# Autodesk Inventor assembly: Total
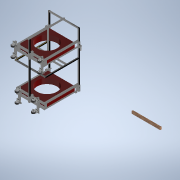
[picture p0: Inventor's stored thumbnail of the model, 180x180]
Saved by Autodesk Inventor 2022 (Build 260153000, 153)
## iProperties
Created: 2022-03-28
Part Number: Total
Document SubType Name: Assembly
Designer: aarco
Author: aarco
## Documents named in this file (14)
- C:\Users\dovalle\OneDrive - ALTER TECHNOLOGY TÜV NORD, S.A.U\Escritorio\IDOM\REV_3\Total.iam
- C:\Users\dovalle\OneDrive - ALTER TECHNOLOGY TÜV NORD, S.A.U\Escritorio\IDOM\REV_3\SoporteBobina_1.iam
- C:\Users\dovalle\OneDrive - ALTER TECHNOLOGY TÜV NORD, S.A.U\Escritorio\IDOM\REV_3\SoporteBobina_2.iam
- C:\Users\dovalle\OneDrive - ALTER TECHNOLOGY TÜV NORD, S.A.U\Escritorio\IDOM\Bobina.ipt
- C:\Users\dovalle\OneDrive - ALTER TECHNOLOGY TÜV NORD, S.A.U\Escritorio\IDOM\REV_2\BPAB 1001 6150.ipt
- C:\Users\dovalle\OneDrive - ALTER TECHNOLOGY TÜV NORD, S.A.U\Escritorio\IDOM\REV_3\Alter\P_3030_1500.ipt
- C:\Users\dovalle\OneDrive - ALTER TECHNOLOGY TÜV NORD, S.A.U\Escritorio\IDOM\REV_3\Alter\P_3030_932.ipt
- C:\Users\dovalle\OneDrive - ALTER TECHNOLOGY TÜV NORD, S.A.U\Escritorio\IDOM\REV_3\Alter\P_3030_883.ipt
- C:\Users\dovalle\OneDrive - ALTER TECHNOLOGY TÜV NORD, S.A.U\Escritorio\IDOM\REV_3\Alter\P_3030_823.ipt
- C:\Users\dovalle\OneDrive - ALTER TECHNOLOGY TÜV NORD, S.A.U\Escritorio\IDOM\REV_3\Alter\Madera.ipt
- C:\Users\dovalle\OneDrive - ALTER TECHNOLOGY TÜV NORD, S.A.U\Escritorio\IDOM\REV_3\Alter\P_3030_735.ipt
- C:\Users\dovalle\OneDrive - ALTER TECHNOLOGY TÜV NORD, S.A.U\Escritorio\IDOM\REV_3\Alter\P_3030_1052.ipt
- C:\Users\dovalle\OneDrive - ALTER TECHNOLOGY TÜV NORD, S.A.U\Escritorio\IDOM\REV_3\BOTTOM_COVER.PRT.ipt
- C:\Users\dovalle\OneDrive - ALTER TECHNOLOGY TÜV NORD, S.A.U\Escritorio\IDOM\psantes.ipt
## Components (29 placed, 13 different names)
1. SoporteBobina_1:1 [sub-assembly] — Coincidencia:1, Nivelación:1, Nivelación:2, Coincidencia:2, Coincidencia:3, Coincidencia:4, Coincidencia:5, Coincidencia:6, Coincidencia:12, Nivelación:7, Nivelación:8, Coincidencia:13, Coincidencia:14, Coincidencia:15, Coincidencia:16, Rigid:12, Rigid:13, Rigid:14
2. SoporteBobina_2:1 [sub-assembly] — Nivelación:1, Nivelación:2, Coincidencia:10, Nivelación:3, Nivelación:4, Coincidencia:11, Nivelación:5, Nivelación:6, Coincidencia:17, Coincidencia:18, Coincidencia:26, Coincidencia:25, Coincidencia:27, Rigid:15, Rigid:16
3. Bobina:2 — Coincidencia:4, Coincidencia:5, Coincidencia:6
4. BPAB 1001 6150:1 — Coincidencia:12, Nivelación:7, Nivelación:8
5. BPAB 1001 6150:2 — Coincidencia:11, Nivelación:5, Nivelación:6
6. BPAB 1001 6150:3 — Coincidencia:10, Nivelación:3, Nivelación:4
7. P_3030_1500:1 — Coincidencia:13, Coincidencia:14, Rígido:2, Slider:8
8. P_3030_1500:2 — Coincidencia:15, Coincidencia:16, Rígido:1, Rigid:18, Slider:9
9. P_3030_1500:3 — Coincidencia:17, Coincidencia:18, Rígido:3
10. P_3030_932:2 — Rígido:1, Rígido:4, Coincidencia:19, Nivelación:13
11. P_3030_932:3 — Rígido:2, Rígido:5, Coincidencia:20, Coincidencia:28
12. P_3030_883:1 — Rígido:3, Rígido:4, Rígido:5
13. Madera:1
14. P_3030_823:2 — Slider:8, Slider:9, Rigid:22, Rigid:23
15. Bobina:3 — Coincidencia:26, Coincidencia:25, Coincidencia:27
16. P_3030_823:3 — Coincidencia:28, Nivelación:13, Rígido:9, Rigid:20, Rigid:21
17. P_3030_735:1 — Rígido:9
18. P_3030_1052:1 — Rigid:19
19. BPAB 1001 6150:4 — Rigid:14
20. BPAB 1001 6150:6 — Rigid:15
21. BPAB 1001 6150:7 — Rigid:12
22. BPAB 1001 6150:8 — Rigid:16
23. BPAB 1001 6150:9 — Rigid:13
24. P_3030_823:4 — Rigid:18, Rigid:19
25. BOTTOM_COVER.PRT:1 — Mate:29, Mate:30, Flush:14
26. psantes:1 — Rigid:21, Mate:29
27. psantes:2 — Rigid:20
28. psantes:3 — Rigid:22, Flush:14
29. psantes:4 — Rigid:23, Mate:30
## Relationships (52: Mate 23, WeldJoint 17, Flush 10, TranslationJoint 2)
- Coincidencia:1 [Mate]: SoporteBobina_1:1
- Nivelación:1 [Flush]: SoporteBobina_1:1 ↔ SoporteBobina_2:1
- Nivelación:2 [Flush]: SoporteBobina_1:1 ↔ SoporteBobina_2:1
- Coincidencia:2 [Mate]: SoporteBobina_1:1
- Coincidencia:3 [Mate]: SoporteBobina_1:1
- Coincidencia:4 [Mate]: SoporteBobina_1:1 ↔ Bobina:2
- Coincidencia:5 [Mate]: SoporteBobina_1:1 ↔ Bobina:2
- Coincidencia:6 [Mate]: SoporteBobina_1:1 ↔ Bobina:2
- Coincidencia:10 [Mate]: SoporteBobina_2:1 ↔ BPAB 1001 6150:3
- Nivelación:3 [Flush]: SoporteBobina_2:1 ↔ BPAB 1001 6150:3
- Nivelación:4 [Flush]: SoporteBobina_2:1 ↔ BPAB 1001 6150:3
- Coincidencia:11 [Mate]: SoporteBobina_2:1 ↔ BPAB 1001 6150:2
- Nivelación:5 [Flush]: SoporteBobina_2:1 ↔ BPAB 1001 6150:2
- Nivelación:6 [Flush]: SoporteBobina_2:1 ↔ BPAB 1001 6150:2
- Coincidencia:12 [Mate]: SoporteBobina_1:1 ↔ BPAB 1001 6150:1
- Nivelación:7 [Flush]: SoporteBobina_1:1 ↔ BPAB 1001 6150:1
- Nivelación:8 [Flush]: SoporteBobina_1:1 ↔ BPAB 1001 6150:1
- Coincidencia:13 [Mate] (1 mm): SoporteBobina_1:1 ↔ P_3030_1500:1
- Coincidencia:14 [Mate] (1 mm): SoporteBobina_1:1 ↔ P_3030_1500:1
- Coincidencia:15 [Mate] (1 mm): SoporteBobina_1:1 ↔ P_3030_1500:2
- Coincidencia:16 [Mate] (1 mm): SoporteBobina_1:1 ↔ P_3030_1500:2
- Coincidencia:17 [Mate] (3 mm): SoporteBobina_2:1 ↔ P_3030_1500:3
- Coincidencia:18 [Mate] (3 mm): SoporteBobina_2:1 ↔ P_3030_1500:3
- Rígido:1 [WeldJoint]: P_3030_1500:2 ↔ P_3030_932:2
- Rígido:2 [WeldJoint]: P_3030_1500:1 ↔ P_3030_932:3
- Rígido:3 [WeldJoint]: P_3030_1500:3 ↔ P_3030_883:1
- Rígido:4 [WeldJoint]: P_3030_932:2 ↔ P_3030_883:1
- Rígido:5 [WeldJoint]: P_3030_932:3 ↔ P_3030_883:1
- Coincidencia:19 [Mate]: P_3030_932:2
- Coincidencia:20 [Mate]: P_3030_932:3
- Slider:8 [TranslationJoint]: P_3030_1500:1 ↔ P_3030_823:2
- Coincidencia:26 [Mate]: SoporteBobina_2:1 ↔ Bobina:3
- Coincidencia:25 [Mate]: SoporteBobina_2:1 ↔ Bobina:3
- Coincidencia:27 [Mate]: SoporteBobina_2:1 ↔ Bobina:3
- Coincidencia:28 [Mate]: P_3030_932:3 ↔ P_3030_823:3
- Nivelación:13 [Flush]: P_3030_932:2 ↔ P_3030_823:3
- Rígido:9 [WeldJoint]: P_3030_823:3 ↔ P_3030_735:1
- Rigid:12 [WeldJoint]: SoporteBobina_1:1 ↔ BPAB 1001 6150:7
- Rigid:13 [WeldJoint]: SoporteBobina_1:1 ↔ BPAB 1001 6150:9
- Rigid:14 [WeldJoint]: SoporteBobina_1:1 ↔ BPAB 1001 6150:4
- Rigid:15 [WeldJoint]: SoporteBobina_2:1 ↔ BPAB 1001 6150:6
- Rigid:16 [WeldJoint]: SoporteBobina_2:1 ↔ BPAB 1001 6150:8
- Rigid:18 [WeldJoint]: P_3030_1500:2 ↔ P_3030_823:4
- Rigid:19 [WeldJoint]: P_3030_1052:1 ↔ P_3030_823:4
- Slider:9 [TranslationJoint]: P_3030_1500:2 ↔ P_3030_823:2
- Rigid:20 [WeldJoint]: P_3030_823:3 ↔ psantes:2
- Rigid:21 [WeldJoint]: P_3030_823:3 ↔ psantes:1
- Rigid:22 [WeldJoint]: P_3030_823:2 ↔ psantes:3
- Rigid:23 [WeldJoint]: P_3030_823:2 ↔ psantes:4
- Mate:29: BOTTOM_COVER.PRT:1 ↔ psantes:1
- Mate:30: BOTTOM_COVER.PRT:1 ↔ psantes:4
- Flush:14: BOTTOM_COVER.PRT:1 ↔ psantes:3
